# Autodesk Inventor assembly: Hopper Linear Guide with endstop
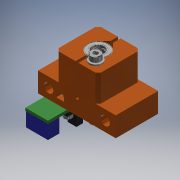
[picture p0: Inventor's stored thumbnail of the model, 180x180]
Saved by Autodesk Inventor 2018 (Build 220112000, 112)
## iProperties
Created: 2017-09-26
Part Number: Hopper Linear Guide with endstop
Document SubType Name: Assembly
Designer: Gabriel Smolnycki
Author: Gabriel Smolnycki
## Documents named in this file (10)
- H:\dev\planb\mechanics\V1INV\Subassemblies\Hopper Linear Guide with endstop.iam
- H:\dev\planb\mechanics\V1INV\Hopper\Hopper Linear Bearing Holder.ipt
- H:\dev\planb\mechanics\V1INV\Hardware\8x25 Linear Bearing (63255K45).ipt
- H:\dev\planb\mechanics\V1INV\Hardware\M4x40 SS SHCS.ipt
- H:\dev\planb\mechanics\V1INV\Hardware\M4 SS Washer.ipt
- H:\dev\planb\mechanics\V1INV\Hardware\M4 SS Nut.ipt
- H:\dev\planb\mechanics\V1INV\Electronics\Endstop.ipt
- H:\dev\planb\mechanics\V1INV\Hardware\M3 SS Washer.ipt
- H:\dev\planb\mechanics\V1INV\Hardware\M3 SS Nut.ipt
- H:\dev\planb\mechanics\V1INV\Hardware\M3x16 SS SHCS.ipt
## Components (17 placed, 9 different names)
1. Hopper Linear Bearing Holder:1 — Mate:1, Insert:1, Insert:3, Mate:2, Insert:5, Mate:3, Insert:6, Insert:7, Insert:10, Insert:17
2. 8x25 Linear Bearing (63255K45):1 — Mate:1, Insert:1
3. M4x40 SS SHCS:1 — Insert:18
4. M4 SS Washer:1 — Insert:3, Insert:4
5. M4 SS Washer:2 — Insert:17, Insert:18
6. M4 SS Nut:1 — Insert:4
7. Endstop:1 — Insert:13, Insert:14, Insert:15, Insert:16
8. M3 SS Washer:1 — Insert:7, Insert:8
9. M3 SS Washer:2 — Insert:8, Insert:9
10. M3 SS Washer:3 — Insert:9, Insert:13
11. M3 SS Washer:4 — Insert:10, Insert:11
12. M3 SS Washer:5 — Insert:11, Insert:12
13. M3 SS Washer:6 — Insert:12, Insert:14
14. M3 SS Nut:1 — Mate:2, Insert:5
15. M3 SS Nut:2 — Mate:3, Insert:6
16. M3x16 SS SHCS:1 — Insert:15
17. M3x16 SS SHCS:2 — Insert:16
## Relationships (20: Insert 17, Mate 3)
- Mate:1: Hopper Linear Bearing Holder:1 ↔ 8x25 Linear Bearing (63255K45):1
- Insert:1: Hopper Linear Bearing Holder:1 ↔ 8x25 Linear Bearing (63255K45):1
- Insert:3: Hopper Linear Bearing Holder:1 ↔ M4 SS Washer:1
- Insert:4: M4 SS Washer:1 ↔ M4 SS Nut:1
- Mate:2: Hopper Linear Bearing Holder:1 ↔ M3 SS Nut:1
- Insert:5: Hopper Linear Bearing Holder:1 ↔ M3 SS Nut:1
- Mate:3: Hopper Linear Bearing Holder:1 ↔ M3 SS Nut:2
- Insert:6: Hopper Linear Bearing Holder:1 ↔ M3 SS Nut:2
- Insert:7: Hopper Linear Bearing Holder:1 ↔ M3 SS Washer:1
- Insert:8: M3 SS Washer:1 ↔ M3 SS Washer:2
- Insert:9: M3 SS Washer:2 ↔ M3 SS Washer:3
- Insert:10: Hopper Linear Bearing Holder:1 ↔ M3 SS Washer:4
- Insert:11: M3 SS Washer:4 ↔ M3 SS Washer:5
- Insert:12: M3 SS Washer:5 ↔ M3 SS Washer:6
- Insert:13: Endstop:1 ↔ M3 SS Washer:3
- Insert:14: Endstop:1 ↔ M3 SS Washer:6
- Insert:15: Endstop:1 ↔ M3x16 SS SHCS:1
- Insert:16: Endstop:1 ↔ M3x16 SS SHCS:2
- Insert:17: Hopper Linear Bearing Holder:1 ↔ M4 SS Washer:2
- Insert:18: M4x40 SS SHCS:1 ↔ M4 SS Washer:2
